# Autodesk Inventor assembly: weld
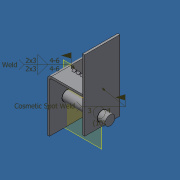
[picture p0: Inventor's stored thumbnail of the model, 180x180]
Saved by Autodesk Inventor 2022.4 (Build 264492010, 492A)
## iProperties
Shininess: 64.0
Length Units: 11269
Angle Units: 11279
Time Units: 11290
Mass Units: 11283
Length Display Precision: 3
Angle Display Precision: 2
Compacted: True
Part Number: weld
Document SubType Name: Weldment
Created: 2002-11-04
Designer: Administrator
Weld Material: Welded Aluminum-6061
Mass: 49.509 g
Surface Area: 320.912 cm^2
Volume: 48.7609 cm^3
Density: 1.01534 g/cm^3
Density: 0.0
Volumn: 0.0
Area: 0.0
PropertySet Name: Model Information
Control State: 0
Master: False
Checked Out: False
CN_MASS: 0.05
Author: Administrator
## Documents named in this file (5)
- U:\Inventor 2022 Training\_Designer Training\Inventor 2022 - Advanced Assembly\Practice Files\weld.iam
- U:\Inventor 2022 Training\_Designer Training\Inventor 2022 - Advanced Assembly\Practice Files\weldangle.ipt
- U:\Inventor 2022 Training\_Designer Training\Inventor 2022 - Advanced Assembly\Practice Files\weldplate.ipt
- U:\Inventor 2022 Training\_Designer Training\Inventor 2022 - Advanced Assembly\Practice Files\gusset.ipt
- U:\Inventor 2022 Training\_Designer Training\Inventor 2022 - Advanced Assembly\Practice Files\pipe.ipt
## Components (4 placed, 4 different names)
1. weldangle:1 — Mate:1, Mate:2, Mate:3, Flush:1, Flush:7, Mate:5
2. weldplate:1 — Mate:1, Mate:2, Mate:3
3. gusset:1 — Flush:2
4. pipe:1 — Flush:7, Mate:5
## Relationships (7: Mate 4, Flush 3)
- Mate:1: weldangle:1 ↔ weldplate:1
- Mate:2 (-50.8 mm): weldangle:1 ↔ weldplate:1
- Mate:3: weldangle:1 ↔ weldplate:1
- Flush:1 (-25.4 mm): weldangle:1
- Flush:2: gusset:1
- Flush:7 (-15 mm): weldangle:1 ↔ pipe:1
- Mate:5: weldangle:1 ↔ pipe:1
